# Autodesk Inventor assembly: top plate assy
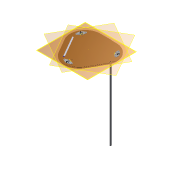
[picture p0: Inventor's stored thumbnail of the model, 180x180]
Saved by Autodesk Inventor 2016 (Build 200138000, 138)
## iProperties
Created: 2016-08-18
Part Number: top plate assy
Document SubType Name: Assembly
Designer: admin
Author: admin
## Documents named in this file (10)
- C:\Users\admin\Desktop\creatablaeD3-이준영 인수인계\1612 3D 도면\top plate assy\top plate assy.iam
- C:\Users\admin\Desktop\creatablaeD3-이준영 인수인계\1612 3D 도면\top plate assy\limit_swich.ipt
- C:\Users\admin\Desktop\creatablaeD3-이준영 인수인계\1612 3D 도면\top plate assy\m3 6 socket_screw.ipt
- C:\Users\admin\Desktop\creatablaeD3-이준영 인수인계\1612 3D 도면\top plate assy\pin 2.5 15.ipt
- C:\Users\admin\Desktop\creatablaeD3-이준영 인수인계\1612 3D 도면\top plate assy\pin 4.ipt
- C:\Users\admin\Desktop\creatablaeD3-이준영 인수인계\1612 3D 도면\top plate assy\plange_bearing.ipt
- C:\Users\admin\Desktop\creatablaeD3-이준영 인수인계\1612 3D 도면\top plate assy\switch_fixer.ipt
- C:\Users\admin\Desktop\creatablaeD3-이준영 인수인계\1612 3D 도면\top plate assy\top_plate.ipt
- C:\Users\admin\Desktop\creatablaeD3-이준영 인수인계\1612 3D 도면\top plate assy\limit_swich_cover.ipt
- C:\Users\admin\Desktop\creatablaeD3-이준영 인수인계\1612 3D 도면\top plate assy\led.ipt
## Components (24 placed, 9 different names)
1. top_plate:1 — Flush:1, Flush:2, Rotational:1, Mate:1, Flush:3, Tangent:1, Tangent:2, Flush:4, Flush:5, Tangent:3, Tangent:4, Mate:2, Mate:5, Mate:6, Angle:1, Mate:9, Mate:10, Mate:11
2. limit_swich_cover:1 — Flush:1, Flush:2
3. led:1 — Mate:9, Mate:10, Mate:11
4. switch_fixer:1 — Mate:5, Mate:6, Mate:7
5. pin 2.5 15:1 — Tangent:1, Tangent:2, Flush:4, Mate:4
6. limit_swich:1 — Mate:2, Mate:3, Mate:4
7. m3 6 socket_screw:1 — Mate:7
8. pin 4:1 — Mate:1, Flush:3
9. plange_bearing:1 — Rotational:1
10. pin 2.5 15:2 — Flush:5, Tangent:3, Tangent:4, Mate:3
11. switch_fixer:2
12. pin 2.5 15:3
13. limit_swich:2
14. m3 6 socket_screw:2
15. pin 4:2
16. plange_bearing:2
17. pin 2.5 15:4
18. switch_fixer:3
19. pin 2.5 15:5
20. limit_swich:3
21. m3 6 socket_screw:3
22. pin 4:3
23. plange_bearing:3
24. pin 2.5 15:6
## Component patterns: (3 elements, first: switch_fixer:1 + pin 2.5 15:1 + limit_swich:1 + m3 6 socket_screw:1 + pin 4:1 + plange_bearing:1 + pin 2.5 15:2)
## Relationships (21: Mate 10, Flush 5, Tangent 4, RevoluteJoint 1, Angle 1)
- Flush:1: top_plate:1 ↔ limit_swich_cover:1
- Flush:2: top_plate:1 ↔ limit_swich_cover:1
- Rotational:1 [RevoluteJoint] (0.1 mm): top_plate:1 ↔ plange_bearing:1
- Mate:1: top_plate:1 ↔ pin 4:1
- Flush:3: top_plate:1 ↔ pin 4:1
- Tangent:1: top_plate:1 ↔ pin 2.5 15:1
- Tangent:2: top_plate:1 ↔ pin 2.5 15:1
- Flush:4: top_plate:1 ↔ pin 2.5 15:1
- Flush:5: top_plate:1 ↔ pin 2.5 15:2
- Tangent:3: top_plate:1 ↔ pin 2.5 15:2
- Tangent:4: top_plate:1 ↔ pin 2.5 15:2
- Mate:2: top_plate:1 ↔ limit_swich:1
- Mate:3: limit_swich:1 ↔ pin 2.5 15:2
- Mate:4: pin 2.5 15:1 ↔ limit_swich:1
- Mate:5: top_plate:1 ↔ switch_fixer:1
- Mate:6: top_plate:1 ↔ switch_fixer:1
- Mate:7: switch_fixer:1 ↔ m3 6 socket_screw:1
- Angle:1 (0 deg): top_plate:1
- Mate:9: top_plate:1 ↔ led:1
- Mate:10 (-2 mm): top_plate:1 ↔ led:1
- Mate:11 (-5 mm): top_plate:1 ↔ led:1
